# Autodesk Inventor assembly: frame
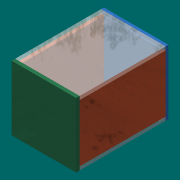
[picture p0: Inventor's stored thumbnail of the model, 180x180]
Saved by Autodesk Inventor 2016 (Build 200138000, 138)
## iProperties
Created: 2015-10-13
Part Number: frame
Document SubType Name: Assembly
Designer: Sawaiz
Author: Sawaiz
## Documents named in this file (6)
- C:\Users\Sawaiz\OneDrive\projects\modularRICH\frame\frame.iam
- C:\Users\Sawaiz\OneDrive\projects\modularRICH\frame\sides.ipt
- C:\Users\Sawaiz\OneDrive\projects\modularRICH\frame\back.iam
- C:\Users\Sawaiz\OneDrive\projects\modularRICH\frame\front.iam
- C:\Users\Sawaiz\OneDrive\projects\modularRICH\frame\topBottom.iam
- C:\Users\Sawaiz\OneDrive\projects\modularRICH\modularRICH.xlsx
## Components (6 placed, 4 different names)
1. back:1 [sub-assembly] — Flush:1, Flush:2, Mate:20
2. front:1 [sub-assembly] — Flush:1, Flush:2, Flush:3, Flush:4, Flush:6, Mate:2, Mate:3, Mate:17, Mate:19
3. topBottom:1 [sub-assembly] — Flush:4, Flush:5, Flush:6, Mate:3
4. topBottom:2 [sub-assembly] — Flush:3, Flush:5, Mate:2, Flush:7, Mate:6, Flush:8, Mate:16, Mate:20
5. sides:1 — Mate:6, Flush:8, Mate:19
6. sides:2 — Flush:7, Mate:16, Mate:17
## Relationships (15: Flush 8, Mate 7)
- Flush:1: back:1 ↔ front:1
- Flush:2: back:1 ↔ front:1
- Flush:3: front:1 ↔ topBottom:2
- Flush:4: front:1 ↔ topBottom:1
- Flush:5: topBottom:1 ↔ topBottom:2
- Flush:6: front:1 ↔ topBottom:1
- Mate:2: front:1 ↔ topBottom:2
- Mate:3: front:1 ↔ topBottom:1
- Flush:7: topBottom:2 ↔ sides:2
- Mate:6: topBottom:2 ↔ sides:1
- Flush:8: topBottom:2 ↔ sides:1
- Mate:16: topBottom:2 ↔ sides:2
- Mate:17: front:1 ↔ sides:2
- Mate:19: front:1 ↔ sides:1
- Mate:20: back:1 ↔ topBottom:2
## Named parameters: acrylicThickness = 6.35 mm, aerogelThickness = 30 mm, height = 101.6 mm, width = 101.6 mm, depth = 152.4 mm, mirrorAngle = 5 deg, detectorWidth = 52 mm, detectorHeight = 52 mm, mirrorThickness = 3.175 mm, fresnelThickness = 0.1 mm, grooveDensity = 100, focalLength = 76.2 mm, ior = 1.49, centerThickness = 1.524 mm, fresnelAngle = 90 deg, fresnelEffectiveDiameter = 76.2 mm, mirrorSuppourtWidth = 38.1 mm, backGrooveBit = 4.8006 mm, sensorHolderWidth = 88.9 mm, sensorHolderSensorWidth = 53.975 mm, sensorHolderSesnorHeight = 53.975 mm, sensorHolderHeight = 88.9 mm, sensorHolderSensorHeight = 53.975 mm, sensorHolderORingGroove = 3.175 mm, sensorHolderORing = 3.175 mm, sensorHolderFlushORingID = 304.8 mm, sensorHolderFlushORing = 3.175 mm, frontBackORingID = 419.1 mm, oRingWidth = 3.175 mm, sensorHolderORingID = 203.2 mm, topBottomHorizontalMirrorGroove = 12.7 mm, backMirrorGroove = 6.35 mm, mirrorGroove = 19.05 mm, compressionPercent = 40, fresnelChamfer = 6.35 mm, mirrorGrooveFillet = 6.35 mm, mirrorGrooveDrill = 6.35 mm, mirrorGrooveMill = 3.175 mm, fresnelMirrorChamfer = 6.35 mm, detectorOpeningHeight = 76.2 mm, detectorOpeningWidth = 76.2 mm
